# Autodesk Inventor assembly: AM14U3+Long+REV1-1
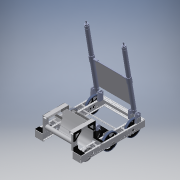
[picture p0: Inventor's stored thumbnail of the model, 180x180]
Saved by Autodesk Inventor 2016 (Build 200138000, 138)
## iProperties
Created: 2015-12-07
Part Number: AM14U3+Long+REV1-1
Description: STEP AP214
Document SubType Name: Assembly
Designer: Douglas
Sending System: SolidWorks 2014
Preprocessor: SwSTEP 2.0
Title: AM14U3 Long REV2.STEP
Revision Number: ANY
## Documents named in this file (7)
- D:\SkyDrive\GitHub\2016-Robot-CAD\Inventor\Chassis\AM14U3+Long+REV1-1.iam
- D:\SkyDrive\GitHub\2016-Robot-CAD\Inventor\PARTS\TMP.ipt
- D:\SkyDrive\GitHub\2016-Robot-CAD\Inventor\PARTS\Lift.iam
- D:\SkyDrive\GitHub\2016-Robot-CAD\Inventor\PARTS\Manipulator.iam
- D:\SkyDrive\GitHub\2016-Robot-CAD\Inventor\Chassis\Left Side.iam
- D:\SkyDrive\GitHub\2016-Robot-CAD\Inventor\Chassis\Right Side.iam
- D:\SkyDrive\GitHub\2016-Robot-CAD\Inventor\PARTS\MiniCIM.ipt
## Components (6 placed, 6 different names)
1. TMP:1
2. Lift:1 [sub-assembly] — Mate:10, Mate:11
3. Manipulator:2 [sub-assembly] — Mate:12, Mate:13, Mate:14
4. Left Side:1 [sub-assembly] — Mate:1, Mate:2, Mate:4, Mate:6, Mate:7, Mate:12, Mate:13, Mate:14
5. Right Side:1 [sub-assembly] — Mate:1, Mate:2, Mate:3, Mate:4, Mate:6, Mate:7, Mate:10, Mate:11
6. MiniCIM:1
## Relationships (11: Mate 11)
- Mate:1: Left Side:1 ↔ Right Side:1
- Mate:2: Left Side:1 ↔ Right Side:1
- Mate:3: Right Side:1
- Mate:4: Left Side:1 ↔ Right Side:1
- Mate:6: Left Side:1 ↔ Right Side:1
- Mate:7: Left Side:1 ↔ Right Side:1
- Mate:10: Lift:1 ↔ Right Side:1
- Mate:11: Lift:1 ↔ Right Side:1
- Mate:12: Manipulator:2 ↔ Left Side:1
- Mate:13: Manipulator:2 ↔ Left Side:1
- Mate:14: Manipulator:2 ↔ Left Side:1
